# Autodesk Inventor assembly: slatHolder_r
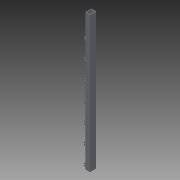
[picture p0: Inventor's stored thumbnail of the model, 180x180]
Saved by Autodesk Inventor 2013 (Build 170138000, 138)
## iProperties
Created: 2013-01-01
Part Number: slatHolder_r
Document SubType Name: Assembly
Designer: Istvan
Author: Istvan
## Documents named in this file (5)
- E:\GitHub\Crown-Fire\CAD\Frame\Table\slatHolder_r.iam
- E:\GitHub\Crown-Fire\CAD\Templates\squareTube1.5x2.ipt
- E:\GitHub\Crown-Fire\CAD\Frame\Table\tableFrameShort.ipt
- E:\GitHub\Crown-Fire\CAD\Frame\Table\slatHolder.ipt
- E:\GitHub\Crown-Fire\CAD\Templates\almRod.5.ipt
## Components (15 placed, 2 different names)
1. tableFrameShort:1 — Tangent:1, Flush:1, Tangent:2, Flush:2
2. slatHolder:1 — Tangent:1, Flush:1, Tangent:3
3. slatHolder:2 — Tangent:2, Flush:2, Tangent:3
4. slatHolder:3
5. slatHolder:4
6. slatHolder:5
7. slatHolder:6
8. slatHolder:7
9. slatHolder:8
10. slatHolder:9
11. slatHolder:10
12. slatHolder:11
13. slatHolder:12
14. slatHolder:13
15. slatHolder:14
## Component patterns: (7 elements, first: slatHolder:1 + slatHolder:2)
## Relationships (5: Tangent 3, Flush 2)
- Tangent:1: tableFrameShort:1 ↔ slatHolder:1
- Flush:1: tableFrameShort:1 ↔ slatHolder:1
- Tangent:2: tableFrameShort:1 ↔ slatHolder:2
- Flush:2: tableFrameShort:1 ↔ slatHolder:2
- Tangent:3 (5.08 mm): slatHolder:1 ↔ slatHolder:2
